# Autodesk Inventor assembly: wheel_base_asm
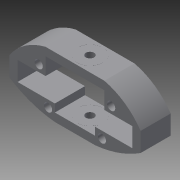
[picture p0: Inventor's stored thumbnail of the model, 180x180]
Saved by Autodesk Inventor 2014 SP1 (Build 180222100, 222)
## iProperties
Created: 2015-07-19
Part Number: wheel_base_asm
Document SubType Name: Assembly
Designer: astralien3000
Author: astralien3000
## Documents named in this file (3)
- C:\Users\astralien3000\Desktop\ceres\meca\v2016\wheel_base_asm.iam
- C:\Users\astralien3000\Desktop\ceres\meca\v2016\wheel_base.ipt
- C:\Users\astralien3000\Desktop\ceres\meca\lib\struct\roulement_6mm.ipt
## Components (3 placed, 2 different names)
1. wheel_base:1 — Placage:1, Affleurement:1, Placage:2, Affleurement:2
2. roulement_6mm:1 — Placage:2, Affleurement:2
3. roulement_6mm:2 — Placage:1, Affleurement:1
## Relationships (4: Mate 2, Flush 2)
- Placage:1 [Mate]: wheel_base:1 ↔ roulement_6mm:2
- Affleurement:1 [Flush]: wheel_base:1 ↔ roulement_6mm:2
- Placage:2 [Mate]: wheel_base:1 ↔ roulement_6mm:1
- Affleurement:2 [Flush]: wheel_base:1 ↔ roulement_6mm:1
